# Autodesk Inventor assembly: Skateboard
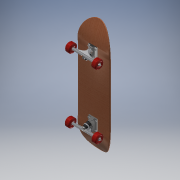
[picture p0: Inventor's stored thumbnail of the model, 180x180]
Saved by Autodesk Inventor 2019 (Build 230136000, 136)
## iProperties
Created: 2020-12-13
Part Number: Skateboard
Document SubType Name: Assembly
Designer: Anass Hamdi
Author: Anass Hamdi
## Documents named in this file (5)
- C:\Users\Anass Hamdi\OneDrive - Vrije Universiteit Brussel\Documenten\Inventor\Anass Hamdi Project\Skateboard.iam
- C:\Users\Anass Hamdi\OneDrive - Vrije Universiteit Brussel\Documenten\Inventor\Anass Hamdi Project\BoardPart.ipt
- C:\Users\Anass Hamdi\OneDrive - Vrije Universiteit Brussel\Documenten\Inventor\Anass Hamdi Project\Trucks.iam
- C:\Users\Anass Hamdi\OneDrive - Vrije Universiteit Brussel\Documenten\Inventor\Anass Hamdi Project\CountersunkBolt.ipt
- C:\Users\Anass Hamdi\OneDrive - Vrije Universiteit Brussel\Documenten\Inventor\Anass Hamdi Project\HexNut.ipt
## Components (19 placed, 4 different names)
1. BoardPart:1 — Rigid:1, Rigid:2, Cylindrical:1, Cylindrical:3, Cylindrical:6, Cylindrical:7, Cylindrical:9, Cylindrical:10, Cylindrical:11, Cylindrical:12
2. Trucks:2 [sub-assembly] — Rigid:1, Cylindrical:13, Cylindrical:14, Cylindrical:15, Cylindrical:16
3. Trucks:3 [sub-assembly] — Rigid:2, Cylindrical:2, Cylindrical:4, Cylindrical:5, Cylindrical:8
4. HexNut_10-32:1 — Cylindrical:2
5. HexNut_10-32:2 — Cylindrical:4
6. HexNut_10-32:3 — Cylindrical:5
7. HexNut_10-32:4 — Cylindrical:8
8. CountersunkBolt:4 — Cylindrical:7
9. CountersunkBolt:2 — Cylindrical:3
10. CountersunkBolt:3 — Cylindrical:6
11. CountersunkBolt:1 — Cylindrical:1
12. CountersunkBolt:5 — Cylindrical:12
13. HexNut_10-32:5 — Cylindrical:14
14. CountersunkBolt:6 — Cylindrical:10
15. HexNut_10-32:6 — Cylindrical:16
16. CountersunkBolt:7 — Cylindrical:11
17. HexNut_10-32:7 — Cylindrical:15
18. CountersunkBolt:8 — Cylindrical:9
19. HexNut_10-32:8 — Cylindrical:13
## Relationships (18: CylindricalJoint 16, WeldJoint 2)
- Rigid:1 [WeldJoint]: BoardPart:1 ↔ Trucks:2
- Rigid:2 [WeldJoint]: BoardPart:1 ↔ Trucks:3
- Cylindrical:1: BoardPart:1 ↔ CountersunkBolt:1
- Cylindrical:2: Trucks:3 ↔ HexNut_10-32:1
- Cylindrical:3: BoardPart:1 ↔ CountersunkBolt:2
- Cylindrical:4: Trucks:3 ↔ HexNut_10-32:2
- Cylindrical:5: Trucks:3 ↔ HexNut_10-32:3
- Cylindrical:6: BoardPart:1 ↔ CountersunkBolt:3
- Cylindrical:7: BoardPart:1 ↔ CountersunkBolt:4
- Cylindrical:8: Trucks:3 ↔ HexNut_10-32:4
- Cylindrical:9: BoardPart:1 ↔ CountersunkBolt:8
- Cylindrical:10: BoardPart:1 ↔ CountersunkBolt:6
- Cylindrical:11: BoardPart:1 ↔ CountersunkBolt:7
- Cylindrical:12: BoardPart:1 ↔ CountersunkBolt:5
- Cylindrical:13: Trucks:2 ↔ HexNut_10-32:8
- Cylindrical:14: Trucks:2 ↔ HexNut_10-32:5
- Cylindrical:15: Trucks:2 ↔ HexNut_10-32:7
- Cylindrical:16: Trucks:2 ↔ HexNut_10-32:6
